# Autodesk Inventor assembly: ASSEMBLY
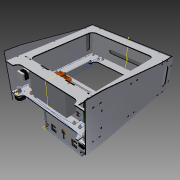
[picture p0: Inventor's stored thumbnail of the model, 180x180]
Saved by Autodesk Inventor 2013 (Build 170138000, 138)
## iProperties
Created: 2014-06-22
Part Number: ASSEMBLY
Document SubType Name: Assembly
Designer: employee
Author: employee
## Documents named in this file (7)
- C:\Users\employee\Desktop\ConceptFORGE\ConceptFORGE\CoreXZ\ASSEMBLY.iam
- C:\Users\employee\Desktop\ConceptFORGE\ConceptFORGE\CoreXZ\FRAME.iam
- C:\Users\employee\Desktop\ConceptFORGE\ConceptFORGE\CoreXZ\GANTRY.iam
- C:\Users\employee\Desktop\ConceptFORGE\ConceptFORGE\CoreXZ\EFFECTOR.iam
- C:\Users\employee\Desktop\ConceptFORGE\ConceptFORGE\CoreXZ\BED.iam
- C:\Users\employee\Desktop\ConceptFORGE\ConceptFORGE\CoreXZ\STRING BED.ipt
- C:\Users\employee\Desktop\ConceptFORGE\ConceptFORGE\CoreXZ\STRING GANTRY.ipt
## Components (6 placed, 6 different names)
1. FRAME:1 [sub-assembly] — Mate:1, Mate:2, Mate:5, Mate:6, Flush:1, Mate:7, Flush:2
2. GANTRY:1 [sub-assembly] — Mate:1, Mate:2, Mate:3, Mate:4, Mate:9
3. EFFECTOR:1 [sub-assembly] — Mate:3, Mate:4, Mate:8, Mate:9
4. BED:1 [sub-assembly] — Mate:5, Mate:6, Mate:7, Mate:8
5. STRING BED:1 — Flush:1
6. STRING GANTRY:1 — Flush:2
## Relationships (11: Mate 9, Flush 2)
- Mate:1: FRAME:1 ↔ GANTRY:1
- Mate:2: FRAME:1 ↔ GANTRY:1
- Mate:3: GANTRY:1 ↔ EFFECTOR:1
- Mate:4: GANTRY:1 ↔ EFFECTOR:1
- Mate:5: FRAME:1 ↔ BED:1
- Mate:6: FRAME:1 ↔ BED:1
- Flush:1: FRAME:1 ↔ STRING BED:1
- Mate:7: FRAME:1 ↔ BED:1
- Mate:8: EFFECTOR:1 ↔ BED:1
- Mate:9: GANTRY:1 ↔ EFFECTOR:1
- Flush:2: FRAME:1 ↔ STRING GANTRY:1
## Named parameters: x = 0 mm, y = 0 mm, z = 0 mm
